# Autodesk Inventor assembly: EnsambleUV-Portatil
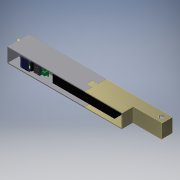
[picture p0: Inventor's stored thumbnail of the model, 180x180]
Saved by Autodesk Inventor 2017 (Build 210142000, 142)
## iProperties
Created: 2021-01-04
Part Number: EnsambleUV-Portatil
Document SubType Name: Assembly
Designer: USUARIO
Author: USUARIO
## Documents named in this file (6)
- D:\Laboratorio\Lampara UV Portatil\2021\Modelo\EnsambleUV-Portatil.iam
- D:\Laboratorio\Lampara UV Portatil\2021\Modelo\Balastro.ipt
- D:\Laboratorio\Lampara UV Portatil\2021\Modelo\SoporteUV.ipt
- D:\Laboratorio\Lampara UV Portatil\2021\Modelo\UV-15W.ipt
- D:\Laboratorio\Lampara UV Portatil\2021\Modelo\SSD1306_i2c.ipt
- D:\Laboratorio\Lampara UV Portatil\2021\Modelo\SoporteUV_Superior.ipt
## Components (5 placed, 5 different names)
1. Balastro:1 — Mate:1, Mate:5
2. SoporteUV:1 — Mate:1, Tangent:1, Angle:1, Mate:2, Mate:3, Mate:4, Mate:5, Mate:6, Mate:7
3. UV-15W:1 — Tangent:1, Angle:1, Mate:2
4. SSD1306_i2c:1 — Mate:3, Mate:4
5. SoporteUV_Superior:1 — Mate:6, Mate:7
## Relationships (9: Mate 7, Tangent 1, Angle 1)
- Mate:1 (1 mm): Balastro:1 ↔ SoporteUV:1
- Tangent:1 (8 mm): SoporteUV:1 ↔ UV-15W:1
- Angle:1 (90 deg): SoporteUV:1 ↔ UV-15W:1
- Mate:2 (-35 mm): SoporteUV:1 ↔ UV-15W:1
- Mate:3 (10 mm): SoporteUV:1 ↔ SSD1306_i2c:1
- Mate:4 (2 mm): SoporteUV:1 ↔ SSD1306_i2c:1
- Mate:5 (2 mm): Balastro:1 ↔ SoporteUV:1
- Mate:6 (0.2 mm): SoporteUV:1 ↔ SoporteUV_Superior:1
- Mate:7: SoporteUV:1 ↔ SoporteUV_Superior:1
